# Autodesk Inventor assembly: ShellyUni
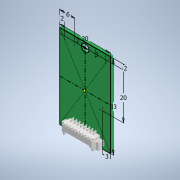
[picture p0: Inventor's stored thumbnail of the model, 180x180]
Saved by Autodesk Inventor 2021 (Build 250183000, 183)
## iProperties
Created: 2021-04-10
Part Number: ShellyUni
Document SubType Name: Assembly
Designer: James
Author: James
## iProperties of the stored document 532610871.ipt
Created: 2019-05-09
Part Number: 532610871
Material: Generic
Document SubType Name: Modeling
Designer: James
Density: 1 g/cm^3
Appearance: Default
Title: 532610871
Author: gga
Revision Number: 8LAST_VERSION
Sending System: PRO/ENGINEER BY PARAMETRIC TECHNOLOGY CORPORATION, 2016010
Preprocessor: PRO/ENGINEER BY PARAMETRIC TECHNOLOGY CORPORATION, 2016010
## Documents named in this file (4)
- **C:\Users\james\Dev\homeprojects\Electronics\XC-0001-Gate_LEDs Rev 3\3D Model\ShellyUni.iam*LocalDocs*xAaaaqdaaAaaaaaaaAaaaazkqTa*532610871.ipt
- C:\Users\james\Dev\homeprojects\Electronics\XC-0001-Gate_LEDs Rev 3\3D Model\ShellyUni.iam
- C:\Users\james\Dev\homeprojects\Electronics\XC-0001-Gate_LEDs Rev 3\3D Model\ShellyUniPCB.ipt
- C:\Users\james\Dev\homeprojects\Electronics\Parts\53261-0871_stp\532610871.stp
## Components (2 placed, 2 different names)
1. ShellyUniPCB:1 — Mate:1, Flush:1, Flush:2
2. 532610871:1 — Mate:1, Flush:1, Flush:2
## Relationships (3: Flush 2, Mate 1)
- Mate:1: ShellyUniPCB:1 ↔ 532610871:1
- Flush:1: ShellyUniPCB:1 ↔ 532610871:1
- Flush:2 (2.425 mm): ShellyUniPCB:1 ↔ 532610871:1
